# Autodesk Inventor assembly: 20X20lift
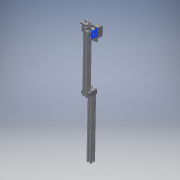
[picture p0: Inventor's stored thumbnail of the model, 180x180]
Saved by Autodesk Inventor 2017 (Build 210142000, 142)
## iProperties
Created: 2017-12-15
Part Number: 20X20lift
Document SubType Name: Assembly
Designer: User
Author: User
## Documents named in this file (11)
- C:\Robotics\CAD\2017-18_CAD\20X20lift.iam
- C:\Robotics\CAD\2017-18_CAD\Prototypes\Sliderfor2020.ipt
- C:\Robotics\CAD\COTSParts\Bosch Extrusion\Bosch 20x20 11.ipt
- C:\Robotics\CAD\2017-18_CAD\Prototypes\ServosSlideforLift.ipt
- C:\Robotics\CAD\COTSParts\Rev\REV-41-1097.ipt
- C:\Robotics\CAD\COTSParts\Actobotics\637 parts\637112\575112.ipt
- C:\Robotics\CAD\COTSParts\Actobotics\637 parts\637112\545420.ipt
- C:\Robotics\CAD\COTSParts\Actobotics\637 parts\637112\535118 assembly.ipt
- C:\Robotics\CAD\COTSParts\Actobotics\637 parts\637112\525123.ipt
- C:\Robotics\CAD\COTSParts\Fasteners\90265A112_18-8 STAINLESS STEEL SHOULDER SCREW.ipt
- C:\Robotics\CAD\COTSParts\Rev\PulleysREV-41-1368.ipt
## Components (17 placed, 10 different names)
1. Sliderfor2020:2 — Mate:30, Mate:31, Mate:32, Mate:33, Insert:28, Insert:29, Flush:13
2. Sliderfor2020:3 — Mate:34, Mate:35, Mate:36, Flush:14, Flush:15, Flush:16
3. Bosch 20x20 11:1 — Mate:30, Mate:40, Mate:41, Mate:42, Flush:14, Flush:15
4. Bosch 20x20 11:2 — Mate:27, Mate:28, Mate:31, Mate:32, Mate:33, Mate:34, Mate:35, Mate:36, Mate:37, Mate:38, Mate:39, Flush:13, Flush:16, Flush:17
5. ServosSlideforLift:1 — Mate:27, Mate:28, Insert:26, Insert:27, Flush:17
6. REV-41-1097:1 — Insert:11, Angle:1, Insert:12
7. 575112:1 — Insert:11, Angle:1, Insert:17, Angle:2
8. 545420:1 — Insert:13, Insert:14, Insert:17, Angle:2, Insert:26, Insert:27
9. 525123:1 — Insert:12
10. 545420:2 — Insert:15, Insert:16
11. 535118 assembly:1 — Insert:13, Insert:14, Insert:15, Insert:16
12. 90265A112_18-8 STAINLESS STEEL SHOULDER SCREW:1 — Insert:28
13. 90265A112_18-8 STAINLESS STEEL SHOULDER SCREW:2 — Insert:24
14. 90265A112_18-8 STAINLESS STEEL SHOULDER SCREW:3 — Insert:23
15. PulleysREV-41-1368:1 — Insert:23, Mate:40, Mate:41, Mate:42
16. PulleysREV-41-1368:2 — Insert:24, Mate:37, Mate:38, Mate:39
17. PulleysREV-41-1368:3 — Insert:29
## Relationships (35: Mate 15, Insert 13, Flush 5, Angle 2)
- Insert:11 (-2.667 mm): REV-41-1097:1 ↔ 575112:1
- Angle:1 (0 deg): REV-41-1097:1 ↔ 575112:1
- Insert:12 (1.905 mm): REV-41-1097:1 ↔ 525123:1
- Insert:13: 545420:1 ↔ 535118 assembly:1
- Insert:14: 545420:1 ↔ 535118 assembly:1
- Insert:15: 545420:2 ↔ 535118 assembly:1
- Insert:16: 545420:2 ↔ 535118 assembly:1
- Insert:17: 575112:1 ↔ 545420:1
- Angle:2 (0 deg): 575112:1 ↔ 545420:1
- Insert:23: 90265A112_18-8 STAINLESS STEEL SHOULDER SCREW:3 ↔ PulleysREV-41-1368:1
- Insert:24: 90265A112_18-8 STAINLESS STEEL SHOULDER SCREW:2 ↔ PulleysREV-41-1368:2
- Mate:27: Bosch 20x20 11:2 ↔ ServosSlideforLift:1
- Mate:28: Bosch 20x20 11:2 ↔ ServosSlideforLift:1
- Insert:26: ServosSlideforLift:1 ↔ 545420:1
- Insert:27: ServosSlideforLift:1 ↔ 545420:1
- Mate:30: Sliderfor2020:2 ↔ Bosch 20x20 11:1
- Mate:31: Sliderfor2020:2 ↔ Bosch 20x20 11:2
- Mate:32 (-10 mm): Sliderfor2020:2 ↔ Bosch 20x20 11:2
- Mate:33 (-10 mm): Sliderfor2020:2 ↔ Bosch 20x20 11:2
- Mate:34: Sliderfor2020:3 ↔ Bosch 20x20 11:2
- Mate:35 (-10 mm): Sliderfor2020:3 ↔ Bosch 20x20 11:2
- Mate:36 (-10 mm): Sliderfor2020:3 ↔ Bosch 20x20 11:2
- Insert:28: Sliderfor2020:2 ↔ 90265A112_18-8 STAINLESS STEEL SHOULDER SCREW:1
- Insert:29: Sliderfor2020:2 ↔ PulleysREV-41-1368:3
- Mate:37: Bosch 20x20 11:2 ↔ PulleysREV-41-1368:2
- Mate:38 (-10 mm): Bosch 20x20 11:2 ↔ PulleysREV-41-1368:2
- Mate:39 (-6 mm): Bosch 20x20 11:2 ↔ PulleysREV-41-1368:2
- Mate:40 (-6 mm): Bosch 20x20 11:1 ↔ PulleysREV-41-1368:1
- Mate:41: Bosch 20x20 11:1 ↔ PulleysREV-41-1368:1
- Mate:42 (-10 mm): Bosch 20x20 11:1 ↔ PulleysREV-41-1368:1
- Flush:13 (3.175 mm): Sliderfor2020:2 ↔ Bosch 20x20 11:2
- Flush:14 (2.4892 mm): Sliderfor2020:3 ↔ Bosch 20x20 11:1
- Flush:15: Sliderfor2020:3 ↔ Bosch 20x20 11:1
- Flush:16: Sliderfor2020:3 ↔ Bosch 20x20 11:2
- Flush:17: Bosch 20x20 11:2 ↔ ServosSlideforLift:1
